# Autodesk Inventor assembly: ASY HPR 300 Frame human
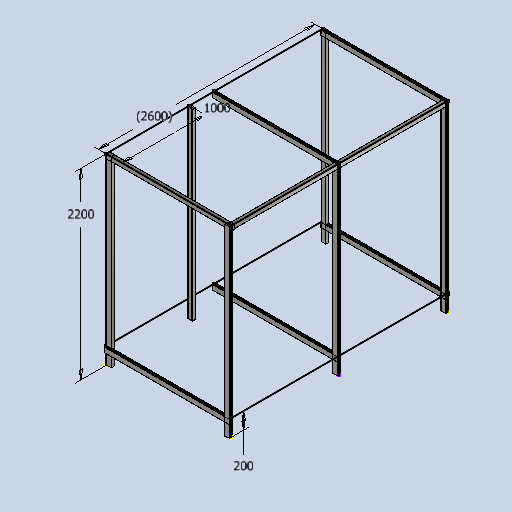
[picture p0: Inventor's stored thumbnail of the model, 512x512]
Saved by Autodesk Inventor 2025.1 (Build 291241020, 241B)
## iProperties
Created: 2024-11-03
Part Number: ASY HPR 300 Frame human
Document SubType Name: Assembly
Designer: admin
_SolveAssemblyDoc: Frame Generator Solve Assembly
_Version: 25.0.0
Author: admin
## Documents named in this file (3)
- C:\Users\user\YandexDisk-badmisterfox\домашниий пк\Inventor\NDM-VOS_powder_hopper\ASY HPR 300 Frame human.iam
- C:\Users\user\YandexDisk-badmisterfox\домашниий пк\Inventor\NDM-VOS_powder_hopper\NDM-VOS dummy staircase.ipt
- C:\Users\user\YandexDisk-badmisterfox\домашниий пк\Inventor\NDM-VOS_powder_hopper\ASY HPR 300 Frame human\Frame\Frame 1730661229799.iam
## Components (2 placed, 2 different names)
1. NDM-VOS dummy staircase:1 — Flush:1, Flush:2, Flush:3
2. Frame 1730661229799:1 [sub-assembly]
## Relationships (3: Flush 3)
- Flush:1: NDM-VOS dummy staircase:1
- Flush:2: NDM-VOS dummy staircase:1
- Flush:3: NDM-VOS dummy staircase:1
